# Autodesk Inventor assembly: stepper_large_all
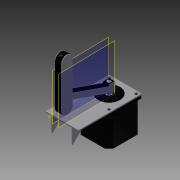
[picture p0: Inventor's stored thumbnail of the model, 180x180]
Saved by Autodesk Inventor 2015 SP1 (Build 190203100, 203)
## iProperties
Created: 2015-04-17
Part Number: stepper_large_all
Document SubType Name: Assembly
Designer: Marcin
Author: Marcin
## Documents named in this file (4)
- C:\Users\Marcin\Documents\Inventor\SynerGolf\motor\stepper_large_all.iam
- C:\Users\Marcin\Documents\Inventor\SynerGolf\motor\stepper_console_large.ipt
- C:\Users\Marcin\Documents\Inventor\SynerGolf\motor\stepper_large.ipt
- C:\Users\Marcin\Documents\Inventor\SynerGolf\club\club_ABS_all.iam
## Components (3 placed, 3 different names)
1. stepper_console_large:1 — Zestawiający:1, Równoległy:1, Zestawiający:2, Kąt:1, Zestawiający:4
2. stepper_large:1 — Kąt:1, Zestawiający:4, Zestawiający:5, Zestawiający:6
3. club_ABS_all:1 [sub-assembly] — Zestawiający:5, Zestawiający:6
## Relationships (7: Mate 5, Flush 1, Angle 1)
- Zestawiający:1 [Mate]: stepper_console_large:1
- Równoległy:1 [Flush]: stepper_console_large:1
- Zestawiający:2 [Mate]: stepper_console_large:1
- Kąt:1 [Angle] (0 deg): stepper_console_large:1 ↔ stepper_large:1
- Zestawiający:4 [Mate]: stepper_console_large:1 ↔ stepper_large:1
- Zestawiający:5 [Mate]: stepper_large:1 ↔ club_ABS_all:1
- Zestawiający:6 [Mate] (3 mm): stepper_large:1 ↔ club_ABS_all:1
